# Autodesk Inventor assembly: Assembly2
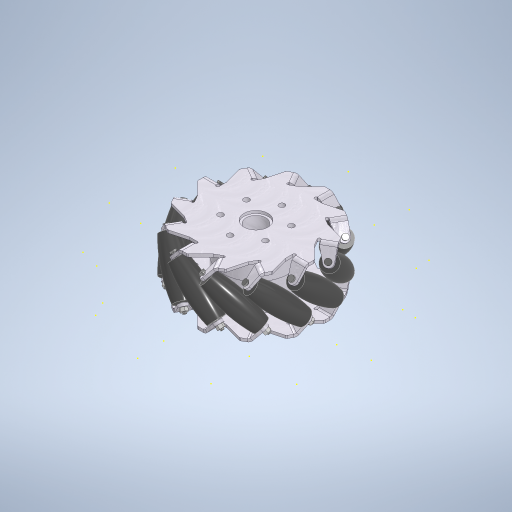
[picture p0: Inventor's stored thumbnail of the model, 512x512]
Saved by Autodesk Inventor 2024 (Build 280153000, 153)
## iProperties
Created: 2023-12-18
Part Number: Assembly2
Document SubType Name: Assembly
Designer: SAHITYA
Author: SAHITYA
## Documents named in this file (5)
- C:\Users\SAHITYA\OneDrive\Documents\Robotics\New folder\Assembly2.iam
- C:\Users\SAHITYA\OneDrive\Documents\Robotics\New folder\Part1.ipt
- C:\Users\SAHITYA\OneDrive\Documents\Robotics\New folder\Part5.ipt
- C:\Users\SAHITYA\OneDrive\Documents\Robotics\New folder\Part7.ipt
- C:\Users\SAHITYA\OneDrive\Documents\Robotics\New folder\Part8.ipt
## Components (38 placed, 4 different names)
1. Part1:1 — Mate:2, Mate:3, Mate:5, Mate:8, Mate:9
2. Part1:2 — Mate:2, Mate:3, Mate:5, Mate:6, Mate:10
3. Part5:1 — Mate:6, Mate:7, Mate:9
4. Part7:1 — Mate:7, Mate:8
5. Part5:2
6. Part7:2
7. Part5:3
8. Part7:3
9. Part5:4
10. Part7:4
11. Part5:5
12. Part7:5
13. Part5:6
14. Part7:6
15. Part5:7
16. Part7:7 — Mate:11
17. Part5:8
18. Part7:8
19. Part5:9
20. Part7:9
21. Part5:10
22. Part7:10
23. Part5:11
24. Part7:11
25. Part5:12
26. Part7:12
27. Part8:1 — Mate:10, Mate:11
28. Part8:2
29. Part8:3
30. Part8:4
31. Part8:5
32. Part8:6
33. Part8:7
34. Part8:8
35. Part8:9
36. Part8:10
37. Part8:11
38. Part8:12
## Component patterns: (12 elements, first: Part5:1 + Part7:1), (12 elements, first: Part8:1)
## Relationships (9: Mate 9)
- Mate:2: Part1:1 ↔ Part1:2
- Mate:3: Part1:1 ↔ Part1:2
- Mate:5: Part1:1 ↔ Part1:2
- Mate:6: Part1:2 ↔ Part5:1
- Mate:7: Part5:1 ↔ Part7:1
- Mate:8 (1 mm): Part1:1 ↔ Part7:1
- Mate:9 (0.5 mm): Part1:1 ↔ Part5:1
- Mate:10: Part1:2 ↔ Part8:1
- Mate:11: Part7:7 ↔ Part8:1
